# Autodesk Inventor assembly: Assembly1
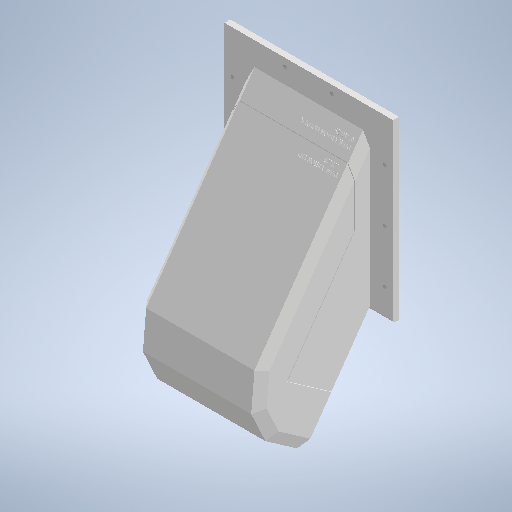
[picture p0: Inventor's stored thumbnail of the model, 512x512]
Saved by Autodesk Inventor 2025.2 (Build 292293000, 293)
## iProperties
Created: 2025-07-18
Part Number: Assembly1
Document SubType Name: Assembly
Designer: mateo
Author: mateo
## Documents named in this file (3)
- C:\GitHub\In-situ-monitoring-of-powder-bed-fusion-additive-manufacturing\system_development\Damascus\v0.3\Hardware\Assembly1.iam
- C:\GitHub\In-situ-monitoring-of-powder-bed-fusion-additive-manufacturing\system_development\Damascus\v0.3\Hardware\cameraholderlid v03.ipt
- C:\GitHub\In-situ-monitoring-of-powder-bed-fusion-additive-manufacturing\system_development\Damascus\v0.3\Hardware\cameraholderbody v03.ipt
## Components (2 placed, 2 different names)
1. cameraholderlid v03:1 — Mate:1, Mate:2
2. cameraholderbody v03:1 — Mate:1, Mate:2
## Relationships (2: Mate 2)
- Mate:1: cameraholderlid v03:1 ↔ cameraholderbody v03:1
- Mate:2: cameraholderlid v03:1 ↔ cameraholderbody v03:1
